# Autodesk Inventor assembly: Sewing Machine Bobbin
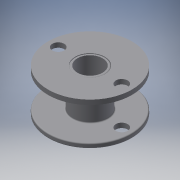
[picture p0: Inventor's stored thumbnail of the model, 180x180]
Saved by Autodesk Inventor 2016 (Build 200138000, 138)
## iProperties
Created: 2015-07-04
Part Number: Sewing Machine Bobbin
Document SubType Name: Assembly
Designer: steele
Author: steele
## Documents named in this file (3)
- C:\snobotics\CAD\robSteele\Steele Sewing Machine Bobbin\Sewing Machine Bobbin.iam
- C:\snobotics\CAD\robSteele\Steele Sewing Machine Bobbin\Steele Sewing Machine Bobbin Base.ipt
- C:\snobotics\CAD\robSteele\Steele Sewing Machine Bobbin\Steele Sewing Machine Bobbin Top.ipt
## Components (2 placed, 2 different names)
1. Steele Sewing Machine Bobbin Base:1 — Mate:1
2. Steele Sewing Machine Bobbin Top:1 — Mate:1
## Relationships (1: Mate 1)
- Mate:1: Steele Sewing Machine Bobbin Base:1 ↔ Steele Sewing Machine Bobbin Top:1
